# Autodesk Inventor assembly: Induction Motor
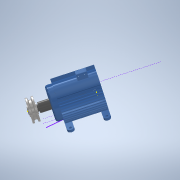
[picture p0: Inventor's stored thumbnail of the model, 180x180]
Saved by Autodesk Inventor 2022 (Build 260153000, 153)
## iProperties
Created: 2021-07-30
Part Number: Induction Motor
Document SubType Name: Assembly
Designer: MOGIRE
Author: MOGIRE
## Documents named in this file (6)
- C:\Users\Mike\Desktop\Mechatronics\Mechatronics 4.1\Manufacturing technology\3phase\3phaseInductionMotor\Induction Motor.iam
- C:\Users\Mike\Desktop\Mechatronics\Mechatronics 4.1\Manufacturing technology\3phase\3phaseInductionMotor\Motor_Frame_.ipt
- C:\Users\MOGIRE\Documents\Manufacturing Technology 4.1\Fan_cover_1.ipt
- C:\Users\Mike\Desktop\Mechatronics\Mechatronics 4.1\Manufacturing technology\3phase\3phaseInductionMotor\Squirrel cage.ipt
- C:\Users\Mike\Desktop\Mechatronics\Mechatronics 4.1\Manufacturing technology\3phase\3phaseInductionMotor\Pulley.ipt
- C:\Users\Mike\Desktop\Mechatronics\Mechatronics 4.1\Manufacturing technology\3phase\3phaseInductionMotor\Fan.ipt
## Components (5 placed, 5 different names)
1. Motor_Frame_:1 — Mate:1, Mate:2, Mate:3, Flush:1, Mate:4
2. Fan_cover_1:1 — Mate:2, Mate:3
3. Squirrel cage:1 — Flush:1, Mate:4, Mate:5, Mate:6, Mate:7, Rotation:9
4. Pulley:1 — Mate:5, Mate:6
5. Fan:1 — Mate:7, Rotation:9
## Relationships (9: Mate 7, Flush 1, RelateRotation 1)
- Mate:1: Motor_Frame_:1
- Mate:2: Motor_Frame_:1 ↔ Fan_cover_1:1
- Mate:3: Motor_Frame_:1 ↔ Fan_cover_1:1
- Flush:1 (50 mm): Motor_Frame_:1 ↔ Squirrel cage:1
- Mate:4: Motor_Frame_:1 ↔ Squirrel cage:1
- Mate:5 (20 mm): Squirrel cage:1 ↔ Pulley:1
- Mate:6: Squirrel cage:1 ↔ Pulley:1
- Mate:7: Squirrel cage:1 ↔ Fan:1
- Rotation:9 [RelateRotation] (1 ul): Squirrel cage:1 ↔ Fan:1
